# Autodesk Inventor assembly: Motor con encaje
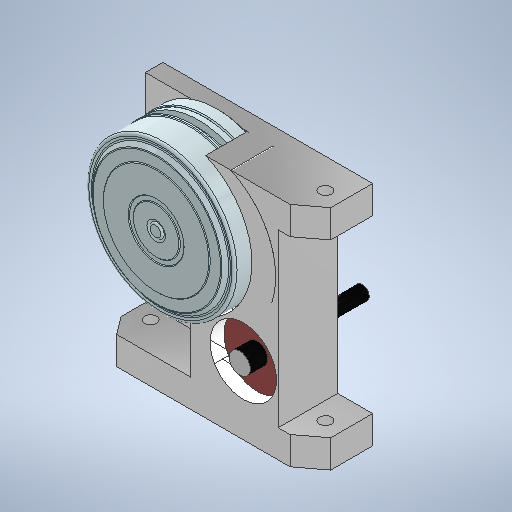
[picture p0: Inventor's stored thumbnail of the model, 512x512]
Saved by Autodesk Inventor 2025.1 (Build 291241000, 241)
## iProperties
Created: 2025-08-29
Part Number: Motor con encaje
Document SubType Name: Assembly
Designer: paeze
Author: paeze
## Documents named in this file (5)
- C:\Users\paeze\Downloads\Base_Ruedas\28_08\Motor con encaje.iam
- C:\Users\paeze\Downloads\Base_Ruedas\28_08\MANCAL DEITADO.ipt
- C:\Users\paeze\Downloads\Base_Ruedas\387266-ec45fl-30w-a-kabel\387266_ec45fl_30w_a_kabel\387266_ec45fl_30w_a_kabel\387266_ec45fl_30w_a_kabel.ipt
- C:\Users\paeze\Downloads\Base_Ruedas\Eje.ipt
- C:\Users\paeze\Downloads\Base_Ruedas\28_08\Ruleman.ipt
## Components (4 placed, 4 different names)
1. MANCAL DEITADO:1 — Rigid:3, Rigid:4
2. 387266_ec45fl_30w_a_kabel:1 — Rigid:3
3. Eje:1 — Cylindrical:1
4. Ruleman:1 — Rigid:4, Cylindrical:1
## Relationships (3: WeldJoint 2, CylindricalJoint 1)
- Rigid:3 [WeldJoint]: MANCAL DEITADO:1 ↔ 387266_ec45fl_30w_a_kabel:1
- Rigid:4 [WeldJoint]: MANCAL DEITADO:1 ↔ Ruleman:1
- Cylindrical:1: Eje:1 ↔ Ruleman:1
